# Autodesk Inventor assembly: original_shutter_hand
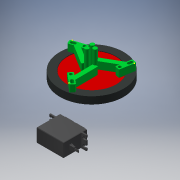
[picture p0: Inventor's stored thumbnail of the model, 180x180]
Saved by Autodesk Inventor 2018 (Build 220112000, 112)
## iProperties
Created: 2019-01-08
Part Number: original_shutter_hand
Material: 一般
Document SubType Name: Assembly
Designer: lowyu
Author: lowyu
## Documents named in this file (6)
- C:\Users\lowyu\Desktop\HAND\シャッターハンド\卒論\originals\original_shutter_hand.iam
- C:\Users\lowyu\Desktop\HAND\シャッターハンド\卒論\originals\parts\fix_plate.ipt
- C:\Users\lowyu\Desktop\HAND\シャッターハンド\卒論\originals\parts\rotate_plate.ipt
- C:\Users\lowyu\Desktop\HAND\シャッターハンド\卒論\originals\parts\finger.ipt
- C:\Users\lowyu\Desktop\HAND\シャッターハンド\卒論\originals\parts\gear_Assembly.iam
- C:\Users\lowyu\Desktop\HAND\シャッターハンド\サーボモータ\body.ipt
## Components (7 placed, 5 different names)
1. fix_plate:1 — メイト:1, メイト:2
2. rotate_plate:1 — メイト:1, メイト:2, メイト:3, メイト:4, メイト:5, メイト:10, メイト:12
3. gear_Assembly:1 [sub-assembly] — メイト:3, メイト:4, メイト:5
4. finger:1
5. finger:2
6. finger:3 — メイト:10, メイト:12
7. body:1
## Relationships (7: Mate 7)
- メイト:1 [Mate]: fix_plate:1 ↔ rotate_plate:1
- メイト:2 [Mate]: fix_plate:1 ↔ rotate_plate:1
- メイト:3 [Mate]: rotate_plate:1 ↔ gear_Assembly:1
- メイト:4 [Mate]: rotate_plate:1 ↔ gear_Assembly:1
- メイト:5 [Mate]: rotate_plate:1 ↔ gear_Assembly:1
- メイト:10 [Mate]: rotate_plate:1 ↔ finger:3
- メイト:12 [Mate]: rotate_plate:1 ↔ finger:3
